# Autodesk Inventor assembly: デフォルト底面
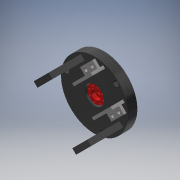
[picture p0: Inventor's stored thumbnail of the model, 180x180]
Saved by Autodesk Inventor 2018 (Build 220112000, 112)
## iProperties
Created: 2018-12-25
Part Number: デフォルト底面
Material: 一般
Document SubType Name: Assembly
Designer: lowyu
Author: lowyu
## Documents named in this file (6)
- C:\Users\lowyu\Desktop\HAND\シャッターハンド\卒論\アセンブリ\デフォルト底面.iam
- C:\Users\lowyu\Desktop\HAND\シャッターハンド\卒論\部品\底面\モータ固定板3.ipt
- C:\Users\lowyu\Desktop\HAND\シャッターハンド\卒論\部品\底面\取付プレート兼　治具.ipt
- C:\Users\lowyu\Desktop\HAND\シャッターハンド\卒論\部品\底面\底面 3盆指.ipt
- C:\Users\lowyu\Desktop\HAND\シャッターハンド\卒論\アセンブリ\デフォルト指アセンブリ.iam
- C:\Users\lowyu\Desktop\HAND\シャッターハンド\卒論\アセンブリ\カム用ボルトアセンブリ.iam
## Components (6 placed, 5 different names)
1. モータ固定板3:1 — メイト:1, メイト:2, メイト:3, メイト:4, メイト:5, メイト:6, メイト:7, メイト:8, メイト:11
2. 取付プレート兼　治具:1 — メイト:4, メイト:5, メイト:6
3. 取付プレート兼　治具:2 — メイト:1, メイト:2, メイト:3
4. 底面 3盆指:1 — メイト:7, メイト:8, メイト:9, メイト:10
5. デフォルト指アセンブリ:1 [sub-assembly] — メイト:9, メイト:10, メイト:12, メイト:13
6. カム用ボルトアセンブリ:1 [sub-assembly] — メイト:11, メイト:12, メイト:13
## Relationships (13: Mate 13)
- メイト:1 [Mate]: モータ固定板3:1 ↔ 取付プレート兼　治具:2
- メイト:2 [Mate]: モータ固定板3:1 ↔ 取付プレート兼　治具:2
- メイト:3 [Mate]: モータ固定板3:1 ↔ 取付プレート兼　治具:2
- メイト:4 [Mate]: モータ固定板3:1 ↔ 取付プレート兼　治具:1
- メイト:5 [Mate]: モータ固定板3:1 ↔ 取付プレート兼　治具:1
- メイト:6 [Mate]: モータ固定板3:1 ↔ 取付プレート兼　治具:1
- メイト:7 [Mate]: モータ固定板3:1 ↔ 底面 3盆指:1
- メイト:8 [Mate]: モータ固定板3:1 ↔ 底面 3盆指:1
- メイト:9 [Mate]: 底面 3盆指:1 ↔ デフォルト指アセンブリ:1
- メイト:10 [Mate]: 底面 3盆指:1 ↔ デフォルト指アセンブリ:1
- メイト:11 [Mate]: モータ固定板3:1 ↔ カム用ボルトアセンブリ:1
- メイト:12 [Mate]: デフォルト指アセンブリ:1 ↔ カム用ボルトアセンブリ:1
- メイト:13 [Mate]: デフォルト指アセンブリ:1 ↔ カム用ボルトアセンブリ:1
